# Autodesk Inventor assembly: Ball Screw balls
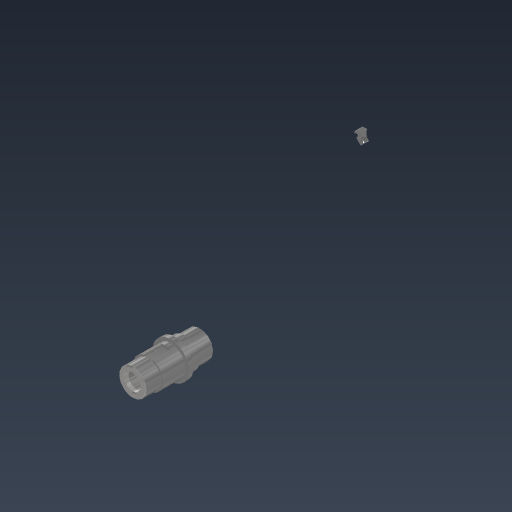
[picture p0: Inventor's stored thumbnail of the model, 512x512]
Saved by Autodesk Inventor 2021 (Build 250183000, 183)
## iProperties
Created: 2020-10-18
Part Number: Ball Screw balls
Document SubType Name: Assembly
Designer: Eugene Tang
Mass: 2585.46 g
Surface Area: 962.441 cm^2
Volume: 323.65 cm^3
Density: 7.98845 g/cm^3
Author: Eugene Tang
## Documents named in this file (5)
- C:\Users\teuge\OneDrive - Curtin University of Technology Australia\Y4S2\DFM\Group Project\CAD\Master\Ball Screw balls.iam
- C:\Users\teuge\OneDrive - Curtin University of Technology Australia\Y4S2\DFM\Group Project\CAD\Master\Ball Screw Balls.ipt
- C:\Users\teuge\OneDrive - Curtin University of Technology Australia\Y4S2\DFM\Group Project\CAD\Master\Ball Screw Nut 1.0.ipt
- C:\Users\teuge\OneDrive - Curtin University of Technology Australia\Y4S2\DFM\Group Project\CAD\Master\Front Returd Mech.ipt
- C:\Users\teuge\OneDrive - Curtin University of Technology Australia\Y4S2\DFM\Group Project\CAD\Master\BallScrewNut Cap.ipt
## Components (6 placed, 4 different names)
1. Ball Screw Nut 1.0:1 — Flush:2, Flush:7, Mate:10, Mate:11, Mate:12, Mate:13, Mate:14, Mate:15, Mate:16
2. Ball Screw Balls:1 — Flush:2, Flush:7
3. BallScrewNut Cap:1 — Mate:12, Mate:13
4. BallScrewNut Cap:2 — Mate:10, Mate:11
5. Front Returd Mech:2 — Mate:14, Mate:15, Mate:16
6. Front Returd Mech:3
## Relationships (9: Mate 7, Flush 2)
- Flush:2: Ball Screw Nut 1.0:1 ↔ Ball Screw Balls:1
- Flush:7: Ball Screw Nut 1.0:1 ↔ Ball Screw Balls:1
- Mate:10: Ball Screw Nut 1.0:1 ↔ BallScrewNut Cap:2
- Mate:11: Ball Screw Nut 1.0:1 ↔ BallScrewNut Cap:2
- Mate:12: Ball Screw Nut 1.0:1 ↔ BallScrewNut Cap:1
- Mate:13: Ball Screw Nut 1.0:1 ↔ BallScrewNut Cap:1
- Mate:14: Ball Screw Nut 1.0:1 ↔ Front Returd Mech:2
- Mate:15: Ball Screw Nut 1.0:1 ↔ Front Returd Mech:2
- Mate:16: Ball Screw Nut 1.0:1 ↔ Front Returd Mech:2
